# Autodesk Inventor assembly: Intake V3
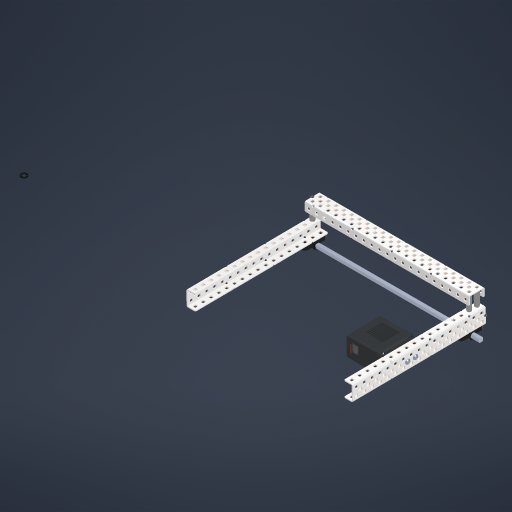
[picture p0: Inventor's stored thumbnail of the model, 512x512]
Saved by Autodesk Inventor 2023.4 (Build 274418000, 418)
## iProperties
Created: 2023-12-16
Part Number: Intake V3
Document SubType Name: Assembly
Designer: diego
Author: diego
## Documents named in this file (12)
- C:\Users\diego\OneDrive\Documents\GitHub\2024-599Z\2024-599Z\Cad\NEW CNC Poly\Intake V3.iam
- C:\Users\diego\OneDrive\Documents\GitHub\2024-599Z\2024-599Z\Cad\Library\VEX-CAD-Inventor-1.4.0\Structure\C Channel\Aluminum 1x2x1\Alu C 1x2x1x21.ipt
- C:\Users\diego\OneDrive\Documents\GitHub\2024-599Z\2024-599Z\Cad\Library\VEX-CAD-Inventor-1.4.0\Structure\Standoff\Standoff 1.00.ipt
- C:\Users\diego\OneDrive\Documents\GitHub\2024-599Z\2024-599Z\Cad\Library\VEX-CAD-Inventor-1.4.0\Structure\Standoff.ipt
- C:\Users\diego\OneDrive\Documents\GitHub\2024-599Z\2024-599Z\Cad\Library\VEX-CAD-Inventor-1.4.0\Structure\C Channel\Aluminum 1x2x1\Alu C 1x2x1x17.ipt
- C:\Users\diego\OneDrive\Documents\GitHub\2024-599Z\2024-599Z\Cad\Library\VEX-CAD-Inventor-1.4.0\Motion\Shaft HS\HS Pillow Bearing Block.ipt
- C:\Users\diego\OneDrive\Documents\GitHub\2024-599Z\2024-599Z\Cad\Library\VEX-CAD-Inventor-1.4.0\Motion\Shaft HS\HS Spacer\HSpacer .0625.ipt
- C:\Users\diego\OneDrive\Documents\GitHub\2024-599Z\2024-599Z\Cad\Library\VEX-CAD-Inventor-1.4.0\Motion\Shaft HS\HS Spacer.ipt
- C:\Users\diego\OneDrive\Documents\GitHub\2024-599Z\2024-599Z\Cad\Library\VEX-CAD-Inventor-1.4.0\Motion\Shaft HS\Shaft HS\Shaft HS 11.0 in.ipt
- C:\Users\diego\OneDrive\Documents\GitHub\2024-599Z\2024-599Z\Cad\Library\VEX-CAD-Inventor-1.4.0\Motion\Shaft HS\Shaft HS.ipt
- C:\Users\diego\OneDrive\Documents\GitHub\2024-599Z\2024-599Z\Cad\Library\VEX-CAD-Inventor-1.4.0\Electronics\Motors with Screws\AluM-StarS.iam
- C:\Users\diego\OneDrive\Documents\GitHub\2024-599Z\2024-599Z\Cad\Library\VEX-CAD-Inventor-1.4.0\Electronics\Motors with Screws.iam
## Components (14 placed, 7 different names)
1. Standoff 1.00:1 — Insert:8, Insert:11
2. Standoff 1.00:2 — Insert:7
3. Standoff 1.00:3 — Insert:6, Insert:13
4. Standoff 1.00:4 — Insert:5, Insert:12
5. Alu C 1x2x1x21:3 — Insert:5, Insert:6, Insert:7, Insert:8
6. HS Pillow Bearing Block:1 — Mate:1, Mate:2, Mate:5, Mate:6, Insert:14
7. HS Pillow Bearing Block:2 — Mate:3, Mate:4, Insert:9, Insert:10
8. HSpacer .0625:1 — Mate:1, Mate:2
9. HSpacer .0625:2 — Mate:3, Mate:4
10. HSpacer .0625:3
11. Shaft HS 11.0 in:1 — Mate:5, Mate:6
12. AluM-StarS:1 [sub-assembly] — Insert:15, Insert:16
13. Alu C 1x2x1x17:1 — Insert:9, Insert:10, Insert:11, Insert:15, Insert:16
14. Alu C 1x2x1x17:2 — Insert:12, Insert:13, Insert:14
## Relationships (18: Insert 12, Mate 6)
- Insert:5: Standoff 1.00:4 ↔ Alu C 1x2x1x21:3
- Insert:6: Standoff 1.00:3 ↔ Alu C 1x2x1x21:3
- Insert:7: Standoff 1.00:2 ↔ Alu C 1x2x1x21:3
- Insert:8: Standoff 1.00:1 ↔ Alu C 1x2x1x21:3
- Mate:1: HS Pillow Bearing Block:1 ↔ HSpacer .0625:1
- Mate:2: HS Pillow Bearing Block:1 ↔ HSpacer .0625:1
- Mate:3: HS Pillow Bearing Block:2 ↔ HSpacer .0625:2
- Mate:4: HS Pillow Bearing Block:2 ↔ HSpacer .0625:2
- Mate:5: HS Pillow Bearing Block:1 ↔ Shaft HS 11.0 in:1
- Mate:6: HS Pillow Bearing Block:1 ↔ Shaft HS 11.0 in:1
- Insert:9: HS Pillow Bearing Block:2 ↔ Alu C 1x2x1x17:1
- Insert:10: HS Pillow Bearing Block:2 ↔ Alu C 1x2x1x17:1
- Insert:11: Standoff 1.00:1 ↔ Alu C 1x2x1x17:1
- Insert:12: Standoff 1.00:4 ↔ Alu C 1x2x1x17:2
- Insert:13: Standoff 1.00:3 ↔ Alu C 1x2x1x17:2
- Insert:14: HS Pillow Bearing Block:1 ↔ Alu C 1x2x1x17:2
- Insert:15: AluM-StarS:1 ↔ Alu C 1x2x1x17:1
- Insert:16: AluM-StarS:1 ↔ Alu C 1x2x1x17:1
